# Autodesk Inventor assembly: Mount_Assembly
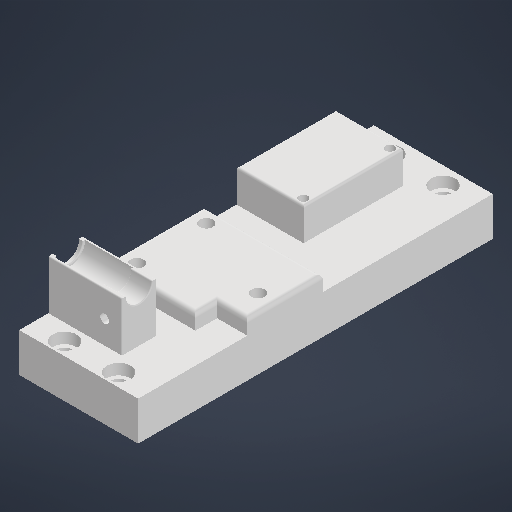
[picture p0: Inventor's stored thumbnail of the model, 512x512]
Saved by Autodesk Inventor 2027.1 (Build 311270010, 270A)
## iProperties
Created: 2026-09-09
Part Number: Mount_Assembly
Document SubType Name: Assembly
Designer: Jacob Parker
Author: Jacob Parker
## Documents named in this file (9)
- C:\Users\Jacob Parker\Documents\GitHub\FUSE-Head\system_development\Pintail\v0.1.3\CAD\Mount_Assembly.iam
- C:\Users\Jacob Parker\Documents\repo\FUSE-Head\system_development\Pintail\V1.1.1\CAD\Sensor_Mount.ipt
- C:\Users\Jacob Parker\Documents\repo\FUSE-Head\system_development\Pintail\V1.1.1\CAD\thermoMETER_mount.ipt
- C:\Users\Jacob Parker\Documents\repo\FUSE-Head\system_development\Pintail\V1.1.1\CAD\Print-head_Mount.ipt
- C:\Users\Jacob Parker\Documents\repo\FUSE-Head\system_development\Pintail\V1.1.1\CAD\optoNCDT_mount.ipt
- C:\Users\Jacob Parker\Documents\repo\FUSE-Head\system_development\Pintail\V1.1.1\CAD\Camera_mount.ipt
- C:\Users\Jacob Parker\Documents\repo\FUSE-Head\system_development\Pintail\V1.1.1\CAD\thermoMETER UC.ipt
- C:\Users\Jacob Parker\Documents\repo\FUSE-Head\system_development\Pintail\V1.1.1\CAD\ILD1x20-500.ipt
- C:\Users\Jacob Parker\Documents\repo\FUSE-Head\system_development\Pintail\V1.1.1\CAD\printer_head.ipt
## Components (8 placed, 8 different names)
1. Sensor_Mount:1 — Mate:1, Mate:2, Mate:3, Flush:1, Flush:2, Flush:3, Flush:4, Flush:5, Mate:4, Flush:6, Mate:5, Angle:1
2. thermoMETER_mount:1 — Mate:1, Flush:1, Rotational:2
3. Print-head_Mount:1 — Mate:2, Flush:2
4. optoNCDT_mount:1 — Mate:3, Flush:3, Mate:5, Rotational:3
5. Camera_mount:1 — Flush:4, Flush:5, Mate:4, Flush:6
6. thermoMETER UC:1 — Rotational:2
7. ILD1x20-500:1 — Rotational:3
8. printer_head:1 — Angle:1
## Relationships (14: Flush 6, Mate 5, RevoluteJoint 2, Angle 1)
- Mate:1: Sensor_Mount:1 ↔ thermoMETER_mount:1
- Mate:2: Sensor_Mount:1 ↔ Print-head_Mount:1
- Mate:3: Sensor_Mount:1 ↔ optoNCDT_mount:1
- Flush:1: Sensor_Mount:1 ↔ thermoMETER_mount:1
- Flush:2: Sensor_Mount:1 ↔ Print-head_Mount:1
- Flush:3: Sensor_Mount:1 ↔ optoNCDT_mount:1
- Flush:4: Sensor_Mount:1 ↔ Camera_mount:1
- Flush:5: Sensor_Mount:1 ↔ Camera_mount:1
- Mate:4: Sensor_Mount:1 ↔ Camera_mount:1
- Flush:6: Sensor_Mount:1 ↔ Camera_mount:1
- Rotational:2 [RevoluteJoint]: thermoMETER_mount:1 ↔ thermoMETER UC:1
- Mate:5: Sensor_Mount:1 ↔ optoNCDT_mount:1
- Rotational:3 [RevoluteJoint]: optoNCDT_mount:1 ↔ ILD1x20-500:1
- Angle:1 (0 deg): Sensor_Mount:1 ↔ printer_head:1
